# Autodesk Inventor assembly: Assembly1
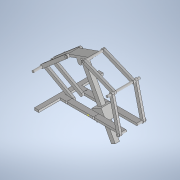
[picture p0: Inventor's stored thumbnail of the model, 180x180]
Saved by Autodesk Inventor 2022 (Build 260153000, 153)
## iProperties
Created: 2021-12-27
Part Number: Assembly1
Document SubType Name: Assembly
Designer: G S SHOURIE
Author: G S SHOURIE
## Documents named in this file (8)
- C:\Users\G S SHOURIE\Desktop\SHOURIE\IMPORTANT STUFF\Ecole Centrale de Nantes\Masters\Studies\Design of Robots\Model\Assembly1.iam
- C:\Users\G S SHOURIE\Desktop\SHOURIE\IMPORTANT STUFF\Ecole Centrale de Nantes\Masters\Studies\Design of Robots\Model\base.ipt
- C:\Users\G S SHOURIE\Desktop\SHOURIE\IMPORTANT STUFF\Ecole Centrale de Nantes\Masters\Studies\Design of Robots\Model\innerLink.ipt
- C:\Users\G S SHOURIE\Desktop\SHOURIE\IMPORTANT STUFF\Ecole Centrale de Nantes\Masters\Studies\Design of Robots\Model\outerLink.ipt
- C:\Users\G S SHOURIE\Desktop\SHOURIE\IMPORTANT STUFF\Ecole Centrale de Nantes\Masters\Studies\Design of Robots\Model\prismaticFulcrum.ipt
- C:\Users\G S SHOURIE\Desktop\SHOURIE\IMPORTANT STUFF\Ecole Centrale de Nantes\Masters\Studies\Design of Robots\Model\endEffector.ipt
- C:\Users\G S SHOURIE\Desktop\SHOURIE\IMPORTANT STUFF\Ecole Centrale de Nantes\Masters\Studies\Design of Robots\Model\prismaticLink.ipt
- C:\Users\G S SHOURIE\Desktop\SHOURIE\IMPORTANT STUFF\Ecole Centrale de Nantes\Masters\Studies\Design of Robots\Model\pin.ipt
## Components (14 placed, 7 different names)
1. base:1 — Mate:1, Mate:2, Mate:3, Mate:4, Mate:6, Mate:7, Mate:8, Mate:9, Mate:11, Mate:12
2. innerLink:2 — Mate:3, Mate:4, Mate:5, Mate:13, Mate:17
3. outerLink:1 — Mate:6, Mate:7, Mate:10, Mate:16, Mate:20, Mate:30, Flush:1
4. outerLink:2 — Mate:8, Mate:9, Mate:10, Mate:15, Mate:19
5. prismaticFulcrum:1 — Mate:11, Mate:12, Mate:27, Mate:28
6. outerLink:3 — Mate:14, Mate:18, Mate:22, Mate:23, Mate:24, Flush:2
7. outerLink:4 — Mate:13, Mate:17, Mate:22
8. outerLink:5 — Mate:15, Mate:19, Mate:21
9. outerLink:7 — Mate:16, Mate:20, Mate:21, Mate:25
10. endEffector:1 — Mate:23, Mate:24, Mate:25, Mate:26
11. prismaticLink:1 — Mate:26, Mate:27, Mate:28
12. pin:1 — Mate:30, Flush:1
13. pin:2 — Mate:29, Flush:2
14. innerLink:1 — Mate:1, Mate:2, Mate:5, Mate:14, Mate:18, Mate:29
## Relationships (32: Mate 30, Flush 2)
- Mate:1: base:1 ↔ innerLink:1
- Mate:2: base:1 ↔ innerLink:1
- Mate:3: base:1 ↔ innerLink:2
- Mate:4: base:1 ↔ innerLink:2
- Mate:5: innerLink:2 ↔ innerLink:1
- Mate:6: base:1 ↔ outerLink:1
- Mate:7: base:1 ↔ outerLink:1
- Mate:8: base:1 ↔ outerLink:2
- Mate:9: base:1 ↔ outerLink:2
- Mate:10: outerLink:1 ↔ outerLink:2
- Mate:11: base:1 ↔ prismaticFulcrum:1
- Mate:12: base:1 ↔ prismaticFulcrum:1
- Mate:13: innerLink:2 ↔ outerLink:4
- Mate:14: outerLink:3 ↔ innerLink:1
- Mate:15: outerLink:2 ↔ outerLink:5
- Mate:16: outerLink:1 ↔ outerLink:7
- Mate:17: innerLink:2 ↔ outerLink:4
- Mate:18: outerLink:3 ↔ innerLink:1
- Mate:19: outerLink:2 ↔ outerLink:5
- Mate:20: outerLink:1 ↔ outerLink:7
- Mate:21: outerLink:5 ↔ outerLink:7
- Mate:22: outerLink:3 ↔ outerLink:4
- Mate:23: outerLink:3 ↔ endEffector:1
- Mate:24: outerLink:3 ↔ endEffector:1
- Mate:25: outerLink:7 ↔ endEffector:1
- Mate:26: endEffector:1 ↔ prismaticLink:1
- Mate:27: prismaticFulcrum:1 ↔ prismaticLink:1
- Mate:28: prismaticFulcrum:1 ↔ prismaticLink:1
- Mate:29: pin:2 ↔ innerLink:1
- Mate:30: outerLink:1 ↔ pin:1
- Flush:1 (12.5 mm): outerLink:1 ↔ pin:1
- Flush:2 (40 mm): outerLink:3 ↔ pin:2
